# Autodesk Inventor assembly: RearWheelNoLogo
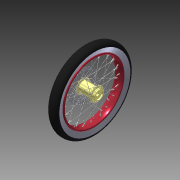
[picture p0: Inventor's stored thumbnail of the model, 180x180]
Saved by Autodesk Inventor 2016 (Build 200138000, 138)
## iProperties
Shininess: 20.0
Length Units: 11269
Angle Units: 11279
Time Units: 11290
Mass Units: 11286
Length Display Precision: 3
Angle Display Precision: 2
Compacted: True
Created: 2001-05-25
Part Number: RearWheelNoLogo
Document SubType Name: Assembly
Designer: Administrator
Density: 0.0
Volumn: 0.0
Area: 0.0
PropertySet Name: Model Information
Control State: 0
Master: False
Checked Out: False
Author: Administrator
## iProperties of the stored document Disk Brake Rotor 230mm.ipt
Created: 2009-08-30
Part Number: Disk Brake Rotor 230mm
Material: SolidWorks Materials|Chrome Stainless Steel|7
Document SubType Name: Modeling
Designer: Yann
Density: 7.8 g/cm^3
Appearance: 229,229,229
Sending System: SolidWorks 2009
Last Author: Administrateur
Last Saved: 2010-11-28
Author: Yann
## Documents named in this file (7)
- **C:\Users\Yann\Documents\GitHub\BIKAIR_CAD\Source\Front_Train\Wheel_spokes\Wheel_spokes.iam*LocalDocs*xCgsrsr1eFgdoe3oxKhlmmklgKg*Disk Brake Rotor 230mm.ipt
- C:\Users\Yann\Documents\GitHub\Bikair_CAD\Source\Front_Train\Wheel_spokes\Wheel_spokes.iam
- C:\Users\Yann\Documents\GitHub\Bikair_CAD\Source\Front_Train\Wheel_spokes\RearHub.ipt
- C:\Users\Yann\Documents\GitHub\Bikair_CAD\Source\Front_Train\Wheel_spokes\ClincherRim2.ipt
- C:\Users\Yann\Documents\GitHub\Bikair_CAD\Source\Front_Train\Wheel_spokes\SpokeRear.ipt
- C:\Users\Yann\Documents\GitHub\Bikair_CAD\Source\Front_Train\Wheel_spokes\wheel_tyre.ipt
- C:\Users\Yann\Documents\GitHub\BIKAIR_CAD\Source\Front_Train\Wheel_spokes\Disk Brake Rotor 230mm.SLDPRT
## Components (44 placed, 5 different names)
1. RearHub:1 — Mate:1, Mate:2, Mate:3, Mate:5, Mate:7, Mate:9
2. ClincherRim2:1 — Mate:1, Mate:3, Mate:4, Mate:6, Mate:8, Mate:10
3. wheel_tyre:1 — Mate:13, Mate:14
4. Disk Brake Rotor 230mm:1 — Mate:15
5. SpokeRear:1 — Mate:2, Mate:4
6. SpokeRear:2 — Mate:5, Mate:6
7. SpokeRear:3 — Mate:7, Mate:8
8. SpokeRear:4 — Mate:9, Mate:10
9. SpokeRear:5
10. SpokeRear:6
11. SpokeRear:7
12. SpokeRear:8
13. SpokeRear:9
14. SpokeRear:10
15. SpokeRear:11
16. SpokeRear:12
17. SpokeRear:13
18. SpokeRear:14
19. SpokeRear:15
20. SpokeRear:16
21. SpokeRear:17
22. SpokeRear:18
23. SpokeRear:19
24. SpokeRear:20
25. SpokeRear:21
26. SpokeRear:22
27. SpokeRear:23
28. SpokeRear:24
29. SpokeRear:25
30. SpokeRear:26
31. SpokeRear:27
32. SpokeRear:28
33. SpokeRear:29
34. SpokeRear:30
35. SpokeRear:31
36. SpokeRear:32
37. SpokeRear:33
38. SpokeRear:34
39. SpokeRear:35
40. SpokeRear:36
41. SpokeRear:37
42. SpokeRear:38
43. SpokeRear:39
44. SpokeRear:40
## Component patterns: (10 elements, first: SpokeRear:1 + SpokeRear:2 + SpokeRear:3 + SpokeRear:4)
## Relationships (13: Mate 13)
- Mate:1: RearHub:1 ↔ ClincherRim2:1
- Mate:2: RearHub:1 ↔ SpokeRear:1
- Mate:3: RearHub:1 ↔ ClincherRim2:1
- Mate:4: ClincherRim2:1 ↔ SpokeRear:1
- Mate:5: RearHub:1 ↔ SpokeRear:2
- Mate:6: ClincherRim2:1 ↔ SpokeRear:2
- Mate:7: RearHub:1 ↔ SpokeRear:3
- Mate:8: ClincherRim2:1 ↔ SpokeRear:3
- Mate:9: RearHub:1 ↔ SpokeRear:4
- Mate:10: ClincherRim2:1 ↔ SpokeRear:4
- Mate:13: wheel_tyre:1
- Mate:14: wheel_tyre:1
- Mate:15: Disk Brake Rotor 230mm:1
